# Autodesk Inventor assembly: Slide rod assembly
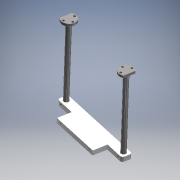
[picture p0: Inventor's stored thumbnail of the model, 180x180]
Saved by Autodesk Inventor 2017 (Build 210142000, 142)
## iProperties
Created: 2016-12-06
Part Number: Slide rod assembly
Document SubType Name: Assembly
Designer: qupec
Author: qupec
## Documents named in this file (3)
- C:\UMD\BPP\ROCKSAT X\star\CAD\Mechanical\Subsystems\Slide Rods\Slide rod assembly.iam
- C:\UMD\BPP\ROCKSAT X\star\CAD\Mechanical\Subsystems\Slide Rods\Slide rod connector.ipt
- C:\UMD\BPP\ROCKSAT X\star\CAD\Mechanical\Subsystems\Slide Rods\slide rod.ipt
## Components (3 placed, 2 different names)
1. Slide rod connector:1 — Mate:1, Mate:11, Mate:12, Flush:1, Flush:2, Mate:18
2. slide rod:1 — Mate:11, Flush:2, Mate:18
3. slide rod:2 — Mate:1, Mate:12, Flush:1
## Relationships (6: Mate 4, Flush 2)
- Mate:1: Slide rod connector:1 ↔ slide rod:2
- Mate:11: Slide rod connector:1 ↔ slide rod:1
- Mate:12: Slide rod connector:1 ↔ slide rod:2
- Flush:1: Slide rod connector:1 ↔ slide rod:2
- Flush:2: Slide rod connector:1 ↔ slide rod:1
- Mate:18: Slide rod connector:1 ↔ slide rod:1
